# Autodesk Inventor assembly: CAD_1
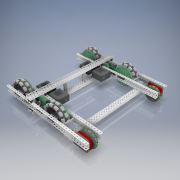
[picture p0: Inventor's stored thumbnail of the model, 180x180]
Saved by Autodesk Inventor 2022 (Build 260153000, 153)
## iProperties
Created: 2021-05-23
Part Number: CAD_1
Document SubType Name: Assembly
Designer: carlo
Author: carlo
## Documents named in this file (25)
- C:\the7dorks.github.io\CAD_1.iam
- C:\the7dorks.github.io\Library 1.2\Motion\Wheels\Omnis\4 Omni, Square.ipt
- C:\the7dorks.github.io\Library 1.2\Structure\C-Channels\Aluminum 1x2x1\1x2x1x35 Aluminum.ipt
- C:\the7dorks.github.io\Library 1.2\Motion\Gears\HS 36T Gear, Circle.ipt
- C:\the7dorks.github.io\Library 1.2\Electronics\Sensors\Optical Shaft Encoder.ipt
- C:\the7dorks.github.io\Library 1.2\Motion\Wheels\Omnis\2.75 Omni - Old.ipt
- C:\the7dorks.github.io\Library 1.2\Electronics\V5 Motor.ipt
- C:\the7dorks.github.io\Tipping Poing Field CAD\Alliance_Mobile_Goal_Red.iam
- C:\the7dorks.github.io\Library 1.2\Motion\Bearing Flat.ipt
- C:\the7dorks.github.io\Library 1.2\Motion\Metal Lock Bar.ipt
- C:\the7dorks.github.io\Library 1.2\Motion\Spacers\Teflon_Washer_275-1025.ipt
- C:\the7dorks.github.io\Library 1.2\Motion\Spacers\Spacer (Nylon), .375 OD\.125 in Grey Spacer.ipt
- C:\the7dorks.github.io\Library 1.2\Structure\Hardware\Bolt 1.5 inch.ipt
- C:\the7dorks.github.io\Library 1.2\Motion\Spacers\Spacer (Nylon), .375 OD\.25 in Grey Spacer.ipt
- C:\the7dorks.github.io\Library 1.2\Structure\Hardware\Nut Thin Nylock.ipt
- C:\the7dorks.github.io\Library 1.2\Motion\Gears\84T Gear.ipt
- C:\the7dorks.github.io\Library 1.2\Structure\Hardware\Bolt 0.5 inch.ipt
- C:\the7dorks.github.io\Library 1.2\Motion\Gears\36T Gear.ipt
- C:\the7dorks.github.io\Library 1.2\Motion\Shaft Collar with Set Screw.ipt
- C:\the7dorks.github.io\Library 1.2\Motion\Spacers\Spacer (Nylon), .375 OD\.5 in Grey Spacer.ipt
- C:\the7dorks.github.io\Library 1.2\Structure\Hardware\Nut Keps.ipt
- C:\the7dorks.github.io\Library 1.2\Structure\Hardware\Standoff 0.5 inch.ipt
- C:\the7dorks.github.io\Library 1.2\Structure\Hardware\Standoff 1.5 inch.ipt
- C:\the7dorks.github.io\Library 1.2\Motion\Shaft Collar with .25 Screw.ipt
- C:\the7dorks.github.io\Library 1.2\Structure\Hardware\Standoff 2.0 inch.ipt
## Components (190 placed, 24 different names)
1. 1x2x1x35 Aluminum:1 — Flush:7, Mate:1, Mate:2, Insert:5, Insert:6, Insert:7, Insert:8, Insert:9, Insert:10, Insert:11, Insert:12, Insert:96, Insert:97, Insert:116, Insert:127, Insert:131, Insert:145, Insert:154, Insert:155, Insert:165, Insert:166, Insert:169, Insert:170, Insert:183, Insert:184, Insert:191, Insert:192, Insert:292, Insert:293
2. 2.75 Omni - Old:1
3. Optical Shaft Encoder:1
4. V5 Motor:1 — Insert:115, Mate:72
5. V5 Motor:2 — Insert:114, Mate:71
6. Alliance_Mobile_Goal_Red:1 [sub-assembly]
7. 1x2x1x35 Aluminum:3 — Insert:100, Insert:101, Insert:102, Insert:103, Insert:114, Mate:71, Insert:115, Mate:72, Insert:136, Insert:137, Insert:146, Insert:147, Insert:148, Insert:149, Insert:167, Insert:168, Insert:171, Insert:172, Insert:181, Insert:182, Insert:193, Insert:194
8. Bearing Flat:1 — Insert:5, Insert:6
9. Bearing Flat:2 — Insert:7, Insert:8
10. Bearing Flat:3 — Insert:9, Insert:10
11. Bearing Flat:4 — Insert:11, Insert:12
12. 84T Gear:1 — Insert:88, Insert:89, Insert:90, Mate:76, Mate:78
13. Metal Lock Bar:14 — Insert:88, Insert:89, Mate:58, Mate:59, Insert:92, Insert:93, Mate:79
14. 4 Omni, Square:7 — Insert:91, Mate:57
15. Teflon_Washer_275-1025:21 — Insert:90, Insert:91
16. Metal Lock Bar:15 — Mate:57, Mate:58, Mate:59, Insert:94, Insert:95, Mate:77
17. Bolt 1.5 inch:1 — Insert:93
18. Bolt 1.5 inch:2 — Insert:92
19. Nut Thin Nylock:11 — Insert:94
20. Nut Thin Nylock:12 — Insert:95
21. Bolt 0.5 inch:1 — Insert:96
22. Bolt 0.5 inch:2 — Insert:97
23. Bearing Flat:6 — Insert:100, Insert:101
24. Bolt 0.5 inch:3 — Insert:102
25. Bolt 0.5 inch:4 — Insert:103
26. 36T Gear:1 — Insert:132, Insert:135
27. Shaft Collar with Set Screw:1 — Insert:117, Mate:76, Mate:77
28. Teflon_Washer_275-1025:25 — Insert:116, Insert:117
29. .25 in Grey Spacer:5 — Mate:78, Mate:79
30. 84T Gear:2
31. Metal Lock Bar:16
32. 4 Omni, Square:8
33. Teflon_Washer_275-1025:26
34. Metal Lock Bar:17
35. Bolt 1.5 inch:3
36. Bolt 1.5 inch:4
37. Nut Thin Nylock:13
38. Nut Thin Nylock:14
39. Shaft Collar with Set Screw:2
40. Teflon_Washer_275-1025:27 — Insert:127
41. .25 in Grey Spacer:6
42. .5 in Grey Spacer:2 — Insert:131, Insert:185
43. Teflon_Washer_275-1025:28 — Insert:132, Insert:188
44. .125 in Grey Spacer:1 — Insert:134, Insert:135
45. Teflon_Washer_275-1025:29 — Insert:133, Insert:134
46. Teflon_Washer_275-1025:30 — Insert:133
47. Bearing Flat:7 — Insert:136, Insert:137
48. 36T Gear:3
49. .5 in Grey Spacer:4 — Insert:145, Insert:186
50. Teflon_Washer_275-1025:31 — Insert:190
51. .125 in Grey Spacer:2
52. Teflon_Washer_275-1025:32
53. Teflon_Washer_275-1025:33
54. Bearing Flat:8 — Insert:146, Insert:147
55. Bolt 1.5 inch:5 — Insert:148
56. Nut Keps:1 — Insert:149, Insert:150
57. Teflon_Washer_275-1025:34 — Insert:150, Insert:151
58. HS 36T Gear, Circle:1 — Insert:151, Insert:159
59. Bearing Flat:9 — Insert:156, Insert:157
60. Standoff 0.5 inch:1 — Insert:155, Insert:156
61. Standoff 0.5 inch:2 — Insert:154, Insert:157
62. .25 in Grey Spacer:9 — Insert:159
63. Teflon_Washer_275-1025:35 — Insert:160
64. Nut Thin Nylock:15 — Insert:160
65. 1x2x1x35 Aluminum:4 — Insert:195, Insert:196, Insert:280, Insert:281, Insert:282, Insert:283
66. 1x2x1x35 Aluminum:5 — Insert:165, Insert:166, Insert:167, Insert:168
67. Nut Thin Nylock:16 — Insert:169
68. Nut Thin Nylock:17 — Insert:171, Insert:173
69. Nut Thin Nylock:18 — Insert:170
70. Nut Thin Nylock:19 — Insert:172, Insert:174
71. Standoff 1.5 inch:1 — Insert:173, Insert:175
72. Standoff 1.5 inch:2 — Insert:174, Insert:176
73. Teflon_Washer_275-1025:36 — Insert:176
74. Teflon_Washer_275-1025:37 — Insert:175
75. Nut Thin Nylock:20 — Insert:182
76. Standoff 1.5 inch:3
77. Teflon_Washer_275-1025:38
78. Nut Thin Nylock:21 — Insert:181
79. Standoff 1.5 inch:4
80. Teflon_Washer_275-1025:39
81. Nut Thin Nylock:22 — Insert:184
82. Nut Thin Nylock:23 — Insert:183
83. Shaft Collar with .25 Screw:1 — Insert:185, Insert:187
84. Shaft Collar with .25 Screw:2 — Insert:186, Insert:189
85. .5 in Grey Spacer:7 — Insert:187, Insert:188
86. .5 in Grey Spacer:8 — Insert:189, Insert:190
87. .5 in Grey Spacer:9 — Insert:191, Insert:195
88. .5 in Grey Spacer:10 — Insert:194
89. .5 in Grey Spacer:11 — Insert:193
90. .5 in Grey Spacer:12 — Insert:192, Insert:196
91. 1x2x1x35 Aluminum:6 — Insert:285
92. V5 Motor:3
93. V5 Motor:4
94. 1x2x1x35 Aluminum:7 — Insert:284
95. Bearing Flat:10
96. Bearing Flat:11
97. Bearing Flat:12
98. Bearing Flat:13
99. 84T Gear:3
100. Metal Lock Bar:18
101. 4 Omni, Square:9
102. Teflon_Washer_275-1025:40
103. Metal Lock Bar:19
104. Bolt 1.5 inch:6
105. Bolt 1.5 inch:7
106. Nut Thin Nylock:24
107. Nut Thin Nylock:25
108. Bolt 0.5 inch:5
109. Bolt 0.5 inch:6
110. Bearing Flat:14
111. Bolt 0.5 inch:7
112. Bolt 0.5 inch:8
113. 36T Gear:4
114. Shaft Collar with Set Screw:3
115. Teflon_Washer_275-1025:41
116. .25 in Grey Spacer:10
117. 84T Gear:4
118. Metal Lock Bar:20
119. 4 Omni, Square:10
120. Teflon_Washer_275-1025:42
121. Metal Lock Bar:21
122. Bolt 1.5 inch:8
123. Bolt 1.5 inch:9
124. Nut Thin Nylock:26
125. Nut Thin Nylock:27
126. Shaft Collar with Set Screw:4
127. Teflon_Washer_275-1025:43
128. .25 in Grey Spacer:11
129. .5 in Grey Spacer:13
130. Teflon_Washer_275-1025:44
131. .125 in Grey Spacer:3
132. Teflon_Washer_275-1025:45
133. Teflon_Washer_275-1025:46
134. Bearing Flat:15
135. 36T Gear:5
136. .5 in Grey Spacer:14
137. Teflon_Washer_275-1025:47
138. .125 in Grey Spacer:4
139. Teflon_Washer_275-1025:48
140. Teflon_Washer_275-1025:49
141. Bearing Flat:16
142. Bolt 1.5 inch:10
143. Nut Keps:2
144. Teflon_Washer_275-1025:50
145. HS 36T Gear, Circle:2
146. Bearing Flat:17
147. Standoff 0.5 inch:3
148. Standoff 0.5 inch:4
149. .25 in Grey Spacer:12
150. Teflon_Washer_275-1025:51
151. Nut Thin Nylock:28
152. Nut Thin Nylock:29
153. Nut Thin Nylock:30
154. Nut Thin Nylock:31
155. Nut Thin Nylock:32
156. Standoff 1.5 inch:5
157. Standoff 1.5 inch:6
158. Teflon_Washer_275-1025:52
159. Teflon_Washer_275-1025:53
160. Nut Thin Nylock:33
161. Standoff 1.5 inch:7
162. Teflon_Washer_275-1025:54
163. Nut Thin Nylock:34
164. Standoff 1.5 inch:8
165. Teflon_Washer_275-1025:55
166. Nut Thin Nylock:35
167. Nut Thin Nylock:36
168. Shaft Collar with .25 Screw:3
169. Shaft Collar with .25 Screw:4
170. .5 in Grey Spacer:15
171. .5 in Grey Spacer:16
172. .5 in Grey Spacer:17 — Insert:283, Insert:285
173. .5 in Grey Spacer:18 — Insert:281, Insert:284
174. .5 in Grey Spacer:19 — Insert:280
175. .5 in Grey Spacer:20 — Insert:282
176. 2.75 Omni - Old:2
177. Optical Shaft Encoder:2
178. 1x2x1x35 Aluminum:8 — Insert:294, Insert:295, Insert:296, Insert:297
179. .5 in Grey Spacer:21 — Insert:293
180. .5 in Grey Spacer:22
181. .5 in Grey Spacer:23
182. .5 in Grey Spacer:24 — Insert:292
183. .5 in Grey Spacer:25
184. .5 in Grey Spacer:26
185. .5 in Grey Spacer:27
186. .5 in Grey Spacer:28
187. Standoff 2.0 inch:1 — Insert:294
188. Standoff 2.0 inch:2 — Insert:295
189. Standoff 2.0 inch:3 — Insert:296
190. Standoff 2.0 inch:4 — Insert:297
## Relationships (235: Insert 194, Mate 34, Flush 7)
- Flush:1 (228.6 mm)
- Flush:2 (-228.6 mm)
- Flush:3 (228.6 mm)
- Flush:4 (-228.6 mm)
- Flush:5 (457.2 mm)
- Flush:6
- Flush:7: 1x2x1x35 Aluminum:1
- Mate:1: 1x2x1x35 Aluminum:1
- Mate:2 (40.386 mm): 1x2x1x35 Aluminum:1
- Insert:5: 1x2x1x35 Aluminum:1 ↔ Bearing Flat:1
- Insert:6: 1x2x1x35 Aluminum:1 ↔ Bearing Flat:1
- Insert:7: 1x2x1x35 Aluminum:1 ↔ Bearing Flat:2
- Insert:8: 1x2x1x35 Aluminum:1 ↔ Bearing Flat:2
- Insert:9: 1x2x1x35 Aluminum:1 ↔ Bearing Flat:3
- Insert:10: 1x2x1x35 Aluminum:1 ↔ Bearing Flat:3
- Insert:11: 1x2x1x35 Aluminum:1 ↔ Bearing Flat:4
- Insert:12: 1x2x1x35 Aluminum:1 ↔ Bearing Flat:4
- Insert:88: 84T Gear:1 ↔ Metal Lock Bar:14
- Insert:89: 84T Gear:1 ↔ Metal Lock Bar:14
- Insert:90: 84T Gear:1 ↔ Teflon_Washer_275-1025:21
- Insert:91: 4 Omni, Square:7 ↔ Teflon_Washer_275-1025:21
- Mate:57: 4 Omni, Square:7 ↔ Metal Lock Bar:15
- Mate:58: Metal Lock Bar:14 ↔ Metal Lock Bar:15
- Mate:59: Metal Lock Bar:14 ↔ Metal Lock Bar:15
- Insert:92: Metal Lock Bar:14 ↔ Bolt 1.5 inch:2
- Insert:93: Metal Lock Bar:14 ↔ Bolt 1.5 inch:1
- Insert:94: Metal Lock Bar:15 ↔ Nut Thin Nylock:11
- Insert:95: Metal Lock Bar:15 ↔ Nut Thin Nylock:12
- Insert:96: 1x2x1x35 Aluminum:1 ↔ Bolt 0.5 inch:1
- Insert:97: 1x2x1x35 Aluminum:1 ↔ Bolt 0.5 inch:2
- Insert:100: 1x2x1x35 Aluminum:3 ↔ Bearing Flat:6
- Insert:101: 1x2x1x35 Aluminum:3 ↔ Bearing Flat:6
- Insert:102: 1x2x1x35 Aluminum:3 ↔ Bolt 0.5 inch:3
- Insert:103: 1x2x1x35 Aluminum:3 ↔ Bolt 0.5 inch:4
- Insert:114: V5 Motor:2 ↔ 1x2x1x35 Aluminum:3
- Mate:71: V5 Motor:2 ↔ 1x2x1x35 Aluminum:3
- Insert:115: V5 Motor:1 ↔ 1x2x1x35 Aluminum:3
- Mate:72: V5 Motor:1 ↔ 1x2x1x35 Aluminum:3
- Insert:116: 1x2x1x35 Aluminum:1 ↔ Teflon_Washer_275-1025:25
- Insert:117: Shaft Collar with Set Screw:1 ↔ Teflon_Washer_275-1025:25
- Mate:76: 84T Gear:1 ↔ Shaft Collar with Set Screw:1
- Mate:77: Metal Lock Bar:15 ↔ Shaft Collar with Set Screw:1
- Mate:78: 84T Gear:1 ↔ .25 in Grey Spacer:5
- Mate:79: Metal Lock Bar:14 ↔ .25 in Grey Spacer:5
- [Insert]: 84T Gear:2 ↔ Metal Lock Bar:16
- [Insert]: 84T Gear:2 ↔ Metal Lock Bar:16
- [Insert]: 84T Gear:2 ↔ Teflon_Washer_275-1025:26
- [Insert]: 4 Omni, Square:8 ↔ Teflon_Washer_275-1025:26
- [Mate]: 4 Omni, Square:8 ↔ Metal Lock Bar:17
- [Mate]: Metal Lock Bar:16 ↔ Metal Lock Bar:17
- [Mate]: Metal Lock Bar:16 ↔ Metal Lock Bar:17
- [Insert]: Metal Lock Bar:16 ↔ Bolt 1.5 inch:4
- [Insert]: Metal Lock Bar:16 ↔ Bolt 1.5 inch:3
- [Insert]: Metal Lock Bar:17 ↔ Nut Thin Nylock:13
- [Insert]: Metal Lock Bar:17 ↔ Nut Thin Nylock:14
- [Insert]: Shaft Collar with Set Screw:2 ↔ Teflon_Washer_275-1025:27
- [Mate]: 84T Gear:2 ↔ Shaft Collar with Set Screw:2
- [Mate]: Metal Lock Bar:17 ↔ Shaft Collar with Set Screw:2
- [Mate]: 84T Gear:2 ↔ .25 in Grey Spacer:6
- [Mate]: Metal Lock Bar:16 ↔ .25 in Grey Spacer:6
- Insert:127: 1x2x1x35 Aluminum:1 ↔ Teflon_Washer_275-1025:27
- Insert:131: 1x2x1x35 Aluminum:1 ↔ .5 in Grey Spacer:2
- Insert:132: 36T Gear:1 ↔ Teflon_Washer_275-1025:28
- Insert:133: Teflon_Washer_275-1025:29 ↔ Teflon_Washer_275-1025:30
- Insert:134: .125 in Grey Spacer:1 ↔ Teflon_Washer_275-1025:29
- Insert:135: 36T Gear:1 ↔ .125 in Grey Spacer:1
- Insert:136: 1x2x1x35 Aluminum:3 ↔ Bearing Flat:7
- Insert:137: 1x2x1x35 Aluminum:3 ↔ Bearing Flat:7
- [Insert]: 36T Gear:3 ↔ Teflon_Washer_275-1025:31
- [Insert]: Teflon_Washer_275-1025:32 ↔ Teflon_Washer_275-1025:33
- [Insert]: .125 in Grey Spacer:2 ↔ Teflon_Washer_275-1025:32
- [Insert]: 36T Gear:3 ↔ .125 in Grey Spacer:2
- Insert:145: 1x2x1x35 Aluminum:1 ↔ .5 in Grey Spacer:4
- Insert:146: 1x2x1x35 Aluminum:3 ↔ Bearing Flat:8
- Insert:147: 1x2x1x35 Aluminum:3 ↔ Bearing Flat:8
- Insert:148: 1x2x1x35 Aluminum:3 ↔ Bolt 1.5 inch:5
- Insert:149: 1x2x1x35 Aluminum:3 ↔ Nut Keps:1
- Insert:150: Nut Keps:1 ↔ Teflon_Washer_275-1025:34
- Insert:151: Teflon_Washer_275-1025:34 ↔ HS 36T Gear, Circle:1
- Insert:154: 1x2x1x35 Aluminum:1 ↔ Standoff 0.5 inch:2
- Insert:155: 1x2x1x35 Aluminum:1 ↔ Standoff 0.5 inch:1
- Insert:156: Bearing Flat:9 ↔ Standoff 0.5 inch:1
- Insert:157: Bearing Flat:9 ↔ Standoff 0.5 inch:2
- [Insert]: .25 in Grey Spacer:9 ↔ Teflon_Washer_275-1025:35
- Insert:159: HS 36T Gear, Circle:1 ↔ .25 in Grey Spacer:9
- Insert:160: Teflon_Washer_275-1025:35 ↔ Nut Thin Nylock:15
- Insert:165: 1x2x1x35 Aluminum:1 ↔ 1x2x1x35 Aluminum:5
- Insert:166: 1x2x1x35 Aluminum:1 ↔ 1x2x1x35 Aluminum:5
- Insert:167: 1x2x1x35 Aluminum:3 ↔ 1x2x1x35 Aluminum:5
- Insert:168: 1x2x1x35 Aluminum:3 ↔ 1x2x1x35 Aluminum:5
- Insert:169: 1x2x1x35 Aluminum:1 ↔ Nut Thin Nylock:16
- Insert:170: 1x2x1x35 Aluminum:1 ↔ Nut Thin Nylock:18
- Insert:171: 1x2x1x35 Aluminum:3 ↔ Nut Thin Nylock:17
- Insert:172: 1x2x1x35 Aluminum:3 ↔ Nut Thin Nylock:19
- Insert:173: Nut Thin Nylock:17 ↔ Standoff 1.5 inch:1
- Insert:174: Nut Thin Nylock:19 ↔ Standoff 1.5 inch:2
- Insert:175: Standoff 1.5 inch:1 ↔ Teflon_Washer_275-1025:37
- Insert:176: Standoff 1.5 inch:2 ↔ Teflon_Washer_275-1025:36
- [Insert]: Nut Thin Nylock:20 ↔ Standoff 1.5 inch:3
- [Insert]: Standoff 1.5 inch:3 ↔ Teflon_Washer_275-1025:38
- [Insert]: Nut Thin Nylock:21 ↔ Standoff 1.5 inch:4
- [Insert]: Standoff 1.5 inch:4 ↔ Teflon_Washer_275-1025:39
- Insert:181: 1x2x1x35 Aluminum:3 ↔ Nut Thin Nylock:21
- Insert:182: 1x2x1x35 Aluminum:3 ↔ Nut Thin Nylock:20
- Insert:183: 1x2x1x35 Aluminum:1 ↔ Nut Thin Nylock:23
- Insert:184: 1x2x1x35 Aluminum:1 ↔ Nut Thin Nylock:22
- Insert:185: .5 in Grey Spacer:2 ↔ Shaft Collar with .25 Screw:1
- Insert:186: .5 in Grey Spacer:4 ↔ Shaft Collar with .25 Screw:2
- Insert:187: Shaft Collar with .25 Screw:1 ↔ .5 in Grey Spacer:7
- Insert:188: Teflon_Washer_275-1025:28 ↔ .5 in Grey Spacer:7
- Insert:189: Shaft Collar with .25 Screw:2 ↔ .5 in Grey Spacer:8
- Insert:190: Teflon_Washer_275-1025:31 ↔ .5 in Grey Spacer:8
- Insert:191: 1x2x1x35 Aluminum:1 ↔ .5 in Grey Spacer:9
- Insert:192: 1x2x1x35 Aluminum:1 ↔ .5 in Grey Spacer:12
- Insert:193: 1x2x1x35 Aluminum:3 ↔ .5 in Grey Spacer:11
- Insert:194: 1x2x1x35 Aluminum:3 ↔ .5 in Grey Spacer:10
- Insert:195: 1x2x1x35 Aluminum:4 ↔ .5 in Grey Spacer:9
- Insert:196: 1x2x1x35 Aluminum:4 ↔ .5 in Grey Spacer:12
- [Insert]: 1x2x1x35 Aluminum:6 ↔ Bearing Flat:10
- [Insert]: 1x2x1x35 Aluminum:6 ↔ Bearing Flat:10
- [Insert]: 1x2x1x35 Aluminum:6 ↔ Bearing Flat:11
- [Insert]: 1x2x1x35 Aluminum:6 ↔ Bearing Flat:11
- [Insert]: 1x2x1x35 Aluminum:6 ↔ Bearing Flat:12
- [Insert]: 1x2x1x35 Aluminum:6 ↔ Bearing Flat:12
- [Insert]: 1x2x1x35 Aluminum:6 ↔ Bearing Flat:13
- [Insert]: 1x2x1x35 Aluminum:6 ↔ Bearing Flat:13
- [Insert]: 84T Gear:3 ↔ Metal Lock Bar:18
- [Insert]: 84T Gear:3 ↔ Metal Lock Bar:18
- [Insert]: 84T Gear:3 ↔ Teflon_Washer_275-1025:40
- [Insert]: 4 Omni, Square:9 ↔ Teflon_Washer_275-1025:40
- [Mate]: 4 Omni, Square:9 ↔ Metal Lock Bar:19
- [Mate]: Metal Lock Bar:18 ↔ Metal Lock Bar:19
- [Mate]: Metal Lock Bar:18 ↔ Metal Lock Bar:19
- [Insert]: Metal Lock Bar:18 ↔ Bolt 1.5 inch:7
- [Insert]: Metal Lock Bar:18 ↔ Bolt 1.5 inch:6
- [Insert]: Metal Lock Bar:19 ↔ Nut Thin Nylock:24
- [Insert]: Metal Lock Bar:19 ↔ Nut Thin Nylock:25
- [Insert]: 1x2x1x35 Aluminum:6 ↔ Bolt 0.5 inch:5
- [Insert]: 1x2x1x35 Aluminum:6 ↔ Bolt 0.5 inch:6
- [Insert]: 1x2x1x35 Aluminum:7 ↔ Bearing Flat:14
- [Insert]: 1x2x1x35 Aluminum:7 ↔ Bearing Flat:14
- [Insert]: 1x2x1x35 Aluminum:7 ↔ Bolt 0.5 inch:7
- [Insert]: 1x2x1x35 Aluminum:7 ↔ Bolt 0.5 inch:8
- [Insert]: V5 Motor:4 ↔ 1x2x1x35 Aluminum:7
- [Mate]: V5 Motor:4 ↔ 1x2x1x35 Aluminum:7
- [Insert]: V5 Motor:3 ↔ 1x2x1x35 Aluminum:7
- [Mate]: V5 Motor:3 ↔ 1x2x1x35 Aluminum:7
- [Insert]: 1x2x1x35 Aluminum:6 ↔ Teflon_Washer_275-1025:41
- [Insert]: Shaft Collar with Set Screw:3 ↔ Teflon_Washer_275-1025:41
- [Mate]: 84T Gear:3 ↔ Shaft Collar with Set Screw:3
- [Mate]: Metal Lock Bar:19 ↔ Shaft Collar with Set Screw:3
- [Mate]: 84T Gear:3 ↔ .25 in Grey Spacer:10
- [Mate]: Metal Lock Bar:18 ↔ .25 in Grey Spacer:10
- [Insert]: 84T Gear:4 ↔ Metal Lock Bar:20
- [Insert]: 84T Gear:4 ↔ Metal Lock Bar:20
- [Insert]: 84T Gear:4 ↔ Teflon_Washer_275-1025:42
- [Insert]: 4 Omni, Square:10 ↔ Teflon_Washer_275-1025:42
- [Mate]: 4 Omni, Square:10 ↔ Metal Lock Bar:21
- [Mate]: Metal Lock Bar:20 ↔ Metal Lock Bar:21
- [Mate]: Metal Lock Bar:20 ↔ Metal Lock Bar:21
- [Insert]: Metal Lock Bar:20 ↔ Bolt 1.5 inch:9
- [Insert]: Metal Lock Bar:20 ↔ Bolt 1.5 inch:8
- [Insert]: Metal Lock Bar:21 ↔ Nut Thin Nylock:26
- [Insert]: Metal Lock Bar:21 ↔ Nut Thin Nylock:27
- [Insert]: Shaft Collar with Set Screw:4 ↔ Teflon_Washer_275-1025:43
- [Mate]: 84T Gear:4 ↔ Shaft Collar with Set Screw:4
- [Mate]: Metal Lock Bar:21 ↔ Shaft Collar with Set Screw:4
- [Mate]: 84T Gear:4 ↔ .25 in Grey Spacer:11
- [Mate]: Metal Lock Bar:20 ↔ .25 in Grey Spacer:11
- [Insert]: 1x2x1x35 Aluminum:6 ↔ Teflon_Washer_275-1025:43
- [Insert]: 1x2x1x35 Aluminum:6 ↔ .5 in Grey Spacer:13
- [Insert]: 36T Gear:4 ↔ Teflon_Washer_275-1025:44
- [Insert]: Teflon_Washer_275-1025:45 ↔ Teflon_Washer_275-1025:46
- [Insert]: .125 in Grey Spacer:3 ↔ Teflon_Washer_275-1025:45
- [Insert]: 36T Gear:4 ↔ .125 in Grey Spacer:3
- [Insert]: 1x2x1x35 Aluminum:7 ↔ Bearing Flat:15
- [Insert]: 1x2x1x35 Aluminum:7 ↔ Bearing Flat:15
- [Insert]: 36T Gear:5 ↔ Teflon_Washer_275-1025:47
- [Insert]: Teflon_Washer_275-1025:48 ↔ Teflon_Washer_275-1025:49
- [Insert]: .125 in Grey Spacer:4 ↔ Teflon_Washer_275-1025:48
- [Insert]: 36T Gear:5 ↔ .125 in Grey Spacer:4
- [Insert]: 1x2x1x35 Aluminum:6 ↔ .5 in Grey Spacer:14
- [Insert]: 1x2x1x35 Aluminum:7 ↔ Bearing Flat:16
- [Insert]: 1x2x1x35 Aluminum:7 ↔ Bearing Flat:16
- [Insert]: 1x2x1x35 Aluminum:7 ↔ Bolt 1.5 inch:10
- [Insert]: 1x2x1x35 Aluminum:7 ↔ Nut Keps:2
- [Insert]: Nut Keps:2 ↔ Teflon_Washer_275-1025:50
- [Insert]: Teflon_Washer_275-1025:50 ↔ HS 36T Gear, Circle:2
- [Insert]: 1x2x1x35 Aluminum:6 ↔ Standoff 0.5 inch:4
- [Insert]: 1x2x1x35 Aluminum:6 ↔ Standoff 0.5 inch:3
- [Insert]: Bearing Flat:17 ↔ Standoff 0.5 inch:3
- [Insert]: Bearing Flat:17 ↔ Standoff 0.5 inch:4
- [Insert]: .25 in Grey Spacer:12 ↔ Teflon_Washer_275-1025:51
- [Insert]: HS 36T Gear, Circle:2 ↔ .25 in Grey Spacer:12
- [Insert]: Teflon_Washer_275-1025:51 ↔ Nut Thin Nylock:28
- [Insert]: 1x2x1x35 Aluminum:6 ↔ Nut Thin Nylock:29
- [Insert]: 1x2x1x35 Aluminum:6 ↔ Nut Thin Nylock:31
- [Insert]: 1x2x1x35 Aluminum:7 ↔ Nut Thin Nylock:30
- [Insert]: 1x2x1x35 Aluminum:7 ↔ Nut Thin Nylock:32
- [Insert]: Nut Thin Nylock:30 ↔ Standoff 1.5 inch:5
- [Insert]: Nut Thin Nylock:32 ↔ Standoff 1.5 inch:6
- [Insert]: Standoff 1.5 inch:5 ↔ Teflon_Washer_275-1025:53
- [Insert]: Standoff 1.5 inch:6 ↔ Teflon_Washer_275-1025:52
- [Insert]: Nut Thin Nylock:33 ↔ Standoff 1.5 inch:7
- [Insert]: Standoff 1.5 inch:7 ↔ Teflon_Washer_275-1025:54
- [Insert]: Nut Thin Nylock:34 ↔ Standoff 1.5 inch:8
- [Insert]: Standoff 1.5 inch:8 ↔ Teflon_Washer_275-1025:55
- [Insert]: 1x2x1x35 Aluminum:7 ↔ Nut Thin Nylock:34
- [Insert]: 1x2x1x35 Aluminum:7 ↔ Nut Thin Nylock:33
- [Insert]: 1x2x1x35 Aluminum:6 ↔ Nut Thin Nylock:36
- [Insert]: 1x2x1x35 Aluminum:6 ↔ Nut Thin Nylock:35
- [Insert]: .5 in Grey Spacer:13 ↔ Shaft Collar with .25 Screw:3
- [Insert]: .5 in Grey Spacer:14 ↔ Shaft Collar with .25 Screw:4
- [Insert]: Shaft Collar with .25 Screw:3 ↔ .5 in Grey Spacer:15
- [Insert]: Teflon_Washer_275-1025:44 ↔ .5 in Grey Spacer:15
- [Insert]: Shaft Collar with .25 Screw:4 ↔ .5 in Grey Spacer:16
- [Insert]: Teflon_Washer_275-1025:47 ↔ .5 in Grey Spacer:16
- Insert:280: 1x2x1x35 Aluminum:4 ↔ .5 in Grey Spacer:19
- Insert:281: 1x2x1x35 Aluminum:4 ↔ .5 in Grey Spacer:18
- Insert:282: 1x2x1x35 Aluminum:4 ↔ .5 in Grey Spacer:20
- Insert:283: 1x2x1x35 Aluminum:4 ↔ .5 in Grey Spacer:17
- Insert:284: 1x2x1x35 Aluminum:7 ↔ .5 in Grey Spacer:18
- Insert:285: 1x2x1x35 Aluminum:6 ↔ .5 in Grey Spacer:17
- [Insert]: 1x2x1x35 Aluminum:8 ↔ .5 in Grey Spacer:21
- [Insert]: 1x2x1x35 Aluminum:8 ↔ .5 in Grey Spacer:24
- [Insert]: 1x2x1x35 Aluminum:8 ↔ .5 in Grey Spacer:27
- [Insert]: 1x2x1x35 Aluminum:8 ↔ .5 in Grey Spacer:26
- [Insert]: 1x2x1x35 Aluminum:8 ↔ .5 in Grey Spacer:28
- [Insert]: 1x2x1x35 Aluminum:8 ↔ .5 in Grey Spacer:25
- Insert:292: 1x2x1x35 Aluminum:1 ↔ .5 in Grey Spacer:24
- Insert:293: 1x2x1x35 Aluminum:1 ↔ .5 in Grey Spacer:21
- Insert:294: 1x2x1x35 Aluminum:8 ↔ Standoff 2.0 inch:1
- Insert:295: 1x2x1x35 Aluminum:8 ↔ Standoff 2.0 inch:2
- Insert:296: 1x2x1x35 Aluminum:8 ↔ Standoff 2.0 inch:3
- Insert:297: 1x2x1x35 Aluminum:8 ↔ Standoff 2.0 inch:4
## Named parameters: d311_d306 = 0 mm, d312_d307 = 0 mm, d313_d309 = 0 mm, d314_d310 = 0 mm, d315_d258 = 0 mm, d316_d259 = 0 mm, d317_d260 = 0 mm, d318_d261 = 0 mm, d319_d262 = 0 mm, d320_d263 = 0 mm, d321_d264 = 0 mm, d322_d300 = 0 mm, d323_d253 = 0 mm, d324_d254 = 0 mm, d325_d256 = 0 mm, d326_d257 = 0 mm, d344_d332 = 0 mm, d345_d333 = 0 mm, d346_d334 = 0 mm, d347_d335 = 0 mm, d364_d330 = 0 mm, d386_d383 = 0 mm, d387_d385 = 0 mm, d388_d383 = 0 mm, d389_d385 = 0 mm, d408_d96 = 0 mm, d409_d97 = 0 mm, d410_d360 = 0 mm, d411_d361 = 0 mm, d412_d362 = 0 mm, d413_d363 = 0 mm, d414_d364_d330 = 0 mm, d415_d365 = 0 mm, d416_d366 = 0 mm, d417_d344_d332 = 0 mm, d418_d345_d333 = 0 mm, d419_d346_d334 = 0 mm, d420_d347_d335 = 0 mm, d421_d350 = 0 mm, d422_d351 = 0 mm, d423_d352 = 0 mm, d424_d353 = 0 mm, d425_d354 = 0 mm, d426_d355 = 0 mm, d427_d356 = 0 mm, d428_d331 = 0 mm, d429_d332 = 0 mm, d430_d333 = 0 mm, d431_d334 = 0 mm, d432_d335 = 0 mm, d433_d336 = 0 mm, d434_d337 = 0 mm, d435_d98 = 0 mm, d436_d99 = 0 mm, d437_d100 = 0 mm, d438_d101 = 0 mm, d439_d102 = 0 mm, d440_d103 = 0 mm, d441_d306 = 0 mm, d442_d307 = 0 mm, d443_d309 = 0 mm, d444_d310 = 0 mm, d445_d311_d306 = 0 mm, d446_d312_d307 = 0 mm, d447_d313_d309 = 0 mm, d448_d314_d310 = 0 mm, d449_d315_d258 = 0 mm, d450_d316_d259 = 0 mm, d451_d317_d260 = 0 mm, d452_d318_d261 = 0 mm, d453_d319_d262 = 0 mm, d454_d320_d263 = 0 mm, d455_d321_d264 = 0 mm, d456_d322_d300 = 0 mm, d457_d323_d253 = 0 mm, d458_d324_d254 = 0 mm, d459_d325_d256 = 0 mm, d460_d326_d257 = 0 mm, d461_d327 = 0 mm, d462_d258 = 0 mm, d463_d259 = 0 mm, d464_d260 = 0 mm, d465_d261 = 0 mm, d466_d262 = 0 mm, d467_d263 = 0 mm, d468_d264 = 0 mm, d469_d266 = 0 mm, d470_d267 = 0 mm, d471_d378 = 0 mm, d472_d379 = 0 mm, d473_d380 = 0 mm, d474_d381 = 0 mm, d475_d382 = 0 mm, d476_d383 = 0 mm, d477_d384 = 0 mm, d478_d385 = 0 mm, d479_d386_d383 = 0 mm, d480_d387_d385 = 0 mm, d481_d388_d383 = 0 mm, d482_d389_d385 = 0 mm, d483_d390 = 0 mm, d484_d391 = 0 mm, d485_d392 = 0 mm, d486_d393 = 0 mm, d487_d394 = 0 mm, d488_d395 = 0 mm, d489_d396 = 0 mm, d490_d295 = 0 mm, d491_d296 = 0 mm, d492_d297 = 0 mm, d493_d298 = 0 mm, d494_d299 = 0 mm, d495_d300 = 0 mm, d496_d272 = 0 mm, d497_d273 = 0 mm, d498_d274 = 0 mm, d499_d275 = 0 mm, d500_d397 = 0 mm, d501_d398 = 0 mm, d502_d399 = 0 mm, d507_d253 = 0 mm, d508_d254 = 0 mm, d509_d256 = 0 mm, d510_d257 = 0 mm, d518_d511 = 0 mm, d519_d512 = 0 mm, d520_d513 = 0 mm, d521_d514 = 0 mm, d522_d406 = 0 mm, d523_d407 = 0 mm
